# Autodesk Inventor assembly: Shift-block
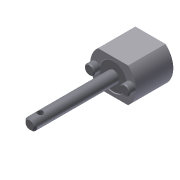
[picture p0: Inventor's stored thumbnail of the model, 180x180]
Saved by Autodesk Inventor 2011 (Build 150239000, 239)
## iProperties
Created: 2011-07-04
Part Number: Shift-block
Document SubType Name: Assembly
Designer: Dan Niemitalo
Mass: 14.2999 g
Surface Area: 39.276 cm^2
Volume: 5.6385 cm^3
Density: 2.53612 g/cm^3
Author: Dan Niemitalo
## Documents named in this file (6)
- H:\Nemo\Documents\Robotics\COTS Parts\Gearboxes\Shifters\Shift Block subassembly.iam
- H:\Nemo\Documents\Robotics\COTS Parts\Gearboxes\Shifters\Shift block.ipt
- H:\Nemo\Documents\Robotics\COTS Parts\Gearboxes\Bearings\Bearing R3.ipt
- H:\Nemo\Documents\Robotics\COTS Parts\Fasteners\4-40 SHCS x500.ipt
- H:\Nemo\Documents\Robotics\COTS Parts\Gearboxes\Shifters\Roll Pin 625x3125.ipt
- H:\Nemo\Documents\Robotics\COTS Parts\Gearboxes\Shifters\Shifting shaft.ipt
## Components (6 placed, 5 different names)
1. Shift block:1 — Insert:1, Insert:2, Insert:3, Tangent:1
2. Bearing R3:1 — Insert:1, Mate:2
3. Shifting shaft:1 — Mate:1, Mate:2
4. Roll Pin 625x3125:1 — Mate:1, Tangent:1, Angle:1
5. 4-40 SHCS x500:2 — Insert:2
6. 4-40 SHCS x500:1 — Insert:3
## Relationships (7: Insert 3, Mate 2, Tangent 1, Angle 1)
- Mate:1: Shifting shaft:1 ↔ Roll Pin 625x3125:1
- Insert:1: Shift block:1 ↔ Bearing R3:1
- Insert:2: Shift block:1 ↔ 4-40 SHCS x500:2
- Insert:3: Shift block:1 ↔ 4-40 SHCS x500:1
- Mate:2: Bearing R3:1 ↔ Shifting shaft:1
- Tangent:1: Shift block:1 ↔ Roll Pin 625x3125:1
- Angle:1 (0 deg): Roll Pin 625x3125:1
